# Autodesk Inventor assembly: Ciąg
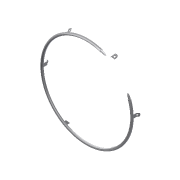
[picture p0: Inventor's stored thumbnail of the model, 180x180]
Saved by Autodesk Inventor 2015 (Build 190159000, 159)
## iProperties
Created: 2016-01-12
Part Number: Ciąg
Document SubType Name: Konstrukcja spawana
Designer: graaapsik
Weld Material: Aluminium 6061-AHC
Author: graaapsik
## Documents named in this file (3)
- C:\Users\EriveltonDell\Documents\Centro Universitário da FEI\Power-Assisted-Wheelchair-master\Power-Assisted-Wheelchair-master\Ciąg.iam
- C:\Users\EriveltonDell\Documents\Centro Universitário da FEI\Power-Assisted-Wheelchair-master\Power-Assisted-Wheelchair-master\Ciąg.ipt
- C:\Users\EriveltonDell\Documents\Centro Universitário da FEI\Power-Assisted-Wheelchair-master\Power-Assisted-Wheelchair-master\Blaszka_do_ciągu.ipt
## Components (7 placed, 2 different names)
1. Ciąg:1 — Równoległy:3
2. Blaszka_do_ciągu:1 — Zestawiający:26, Równoległy:2, Równoległy:3
3. Blaszka_do_ciągu:7
4. Blaszka_do_ciągu:8
5. Blaszka_do_ciągu:9
6. Blaszka_do_ciągu:10
7. Blaszka_do_ciągu:11
## Component patterns: (6 elements, first: Blaszka_do_ciągu:1)
## Relationships (3: Flush 2, Mate 1)
- Zestawiający:26 [Mate] (-10 mm): Blaszka_do_ciągu:1
- Równoległy:2 [Flush] (-251.25 mm): Blaszka_do_ciągu:1
- Równoległy:3 [Flush] (15 mm): Ciąg:1 ↔ Blaszka_do_ciągu:1
